# Autodesk Inventor assembly: 分析
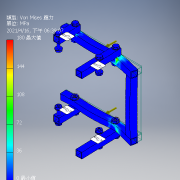
[picture p0: Inventor's stored thumbnail of the model, 180x180]
Saved by Autodesk Inventor 2019 (Build 230136000, 136)
## iProperties
Created: 2019-05-06
Part Number: 分析
Document SubType Name: Assembly
Designer: D03
Author: D03
## Documents named in this file (14)
- C:\Users\user\Desktop\分析.iam
- C:\Users\user\Desktop\新增資料夾\4.ipt
- C:\Users\user\Desktop\新增資料夾\3.ipt
- C:\Users\user\Desktop\新增資料夾\9.ipt
- C:\Users\user\Desktop\新增資料夾\CNS 150 - A - 2.2.ipt
- C:\Users\user\Desktop\新增資料夾\CNS 3128 - M 2 x 0.4.ipt
- C:\Users\user\Desktop\新增資料夾\CNS 3121 - M2 x 12.ipt
- C:\Users\user\Desktop\新增資料夾\2-1.ipt
- C:\Users\user\Desktop\分析\AIP\FEA\dksv0cvts.fins
- C:\Users\user\Desktop\分析\AIP\FEA\dksv0cvts.fsat
- C:\Users\user\Desktop\分析\AIP\FEA\dksv0cvuo.ftes
- C:\Users\user\Desktop\分析\AIP\FEA\dksv0cvuo.fwiz
- C:\Users\user\Desktop\分析\AIP\FEA\dksv0cvz4.fmsh
- C:\Users\user\Desktop\分析\AIP\FEA\dksv0cw00.fres
## Components (39 placed, 7 different names)
1. 3:1 — 插入:6, 插入:10, 插入:13, 插入:24, 貼合:47, 對稱:1, 齊平:22, 齊平:23
2. 3:2 — 插入:7, 插入:8, 插入:20, 插入:23, 貼合:48, 齊平:15, 齊平:16, 對稱:1
3. 4:1 — 插入:7, 插入:18, 插入:19
4. 4:2 — 插入:6, 插入:12, 插入:15
5. 9:1 — 插入:8, 插入:16, 插入:17
6. 9:2 — 插入:10, 插入:26, 插入:27
7. CNS 150 - A - 2.2:1 — 插入:15, 插入:50
8. CNS 150 - A - 2.2:2 — 插入:12, 插入:51
9. CNS 150 - A - 2.2:3 — 插入:24, 插入:36
10. CNS 150 - A - 2.2:4 — 插入:38
11. CNS 150 - A - 2.2:5 — 插入:20, 插入:40
12. CNS 150 - A - 2.2:6 — 插入:41
13. CNS 150 - A - 2.2:7 — 插入:19, 插入:52
14. CNS 150 - A - 2.2:8 — 插入:18, 插入:53
15. CNS 150 - A - 2.2:9 — 插入:26, 插入:48
16. CNS 150 - A - 2.2:10 — 插入:39
17. CNS 150 - A - 2.2:11 — 插入:27, 插入:49
18. CNS 150 - A - 2.2:12 — 插入:13, 插入:37
19. CNS 150 - A - 2.2:13 — 插入:23, 插入:43
20. CNS 150 - A - 2.2:14 — 插入:42
21. CNS 150 - A - 2.2:15 — 插入:17, 插入:54
22. CNS 150 - A - 2.2:16 — 插入:16, 插入:55
23. CNS 3128 - M 2 x 0.4:2 — 插入:39
24. CNS 3128 - M 2 x 0.4:3 — 插入:38
25. CNS 3128 - M 2 x 0.4:4 — 插入:37
26. CNS 3128 - M 2 x 0.4:5 — 插入:36
27. CNS 3128 - M 2 x 0.4:6 — 插入:42
28. CNS 3128 - M 2 x 0.4:7 — 插入:41
29. CNS 3128 - M 2 x 0.4:8 — 插入:43
30. CNS 3128 - M 2 x 0.4:9 — 插入:40
31. CNS 3121 - M2 x 12:1 — 插入:55
32. CNS 3121 - M2 x 12:2 — 插入:54
33. CNS 3121 - M2 x 12:3 — 插入:53
34. CNS 3121 - M2 x 12:4 — 插入:52
35. CNS 3121 - M2 x 12:5 — 插入:50
36. CNS 3121 - M2 x 12:6 — 插入:51
37. CNS 3121 - M2 x 12:7 — 插入:49
38. CNS 3121 - M2 x 12:8 — 插入:48
39. 2-1:2 — 貼合:47, 貼合:48, 齊平:15, 齊平:16, 齊平:22, 齊平:23, 齊平:26
## Relationships (47: Insert 32, Mate 9, Flush 5, Symmetry 1)
- 插入:6 [Insert]: 3:1 ↔ 4:2
- 插入:7 [Insert]: 3:2 ↔ 4:1
- 貼合:24 [Mate]
- 插入:8 [Insert]: 3:2 ↔ 9:1
- 插入:10 [Insert]: 3:1 ↔ 9:2
- 插入:12 [Insert]: 4:2 ↔ CNS 150 - A - 2.2:2
- 插入:13 [Insert]: 3:1 ↔ CNS 150 - A - 2.2:12
- 插入:15 [Insert]: 4:2 ↔ CNS 150 - A - 2.2:1
- 插入:16 [Insert]: 9:1 ↔ CNS 150 - A - 2.2:16
- 插入:17 [Insert]: 9:1 ↔ CNS 150 - A - 2.2:15
- 插入:18 [Insert]: 4:1 ↔ CNS 150 - A - 2.2:8
- 插入:19 [Insert]: 4:1 ↔ CNS 150 - A - 2.2:7
- 插入:20 [Insert]: 3:2 ↔ CNS 150 - A - 2.2:5
- 插入:23 [Insert]: 3:2 ↔ CNS 150 - A - 2.2:13
- 插入:24 [Insert]: 3:1 ↔ CNS 150 - A - 2.2:3
- 插入:26 [Insert]: 9:2 ↔ CNS 150 - A - 2.2:9
- 插入:27 [Insert]: 9:2 ↔ CNS 150 - A - 2.2:11
- 插入:36 [Insert]: CNS 150 - A - 2.2:3 ↔ CNS 3128 - M 2 x 0.4:5
- 插入:37 [Insert]: CNS 150 - A - 2.2:12 ↔ CNS 3128 - M 2 x 0.4:4
- 插入:38 [Insert]: CNS 150 - A - 2.2:4 ↔ CNS 3128 - M 2 x 0.4:3
- 插入:39 [Insert]: CNS 150 - A - 2.2:10 ↔ CNS 3128 - M 2 x 0.4:2
- 插入:40 [Insert]: CNS 150 - A - 2.2:5 ↔ CNS 3128 - M 2 x 0.4:9
- 插入:41 [Insert]: CNS 150 - A - 2.2:6 ↔ CNS 3128 - M 2 x 0.4:7
- 插入:42 [Insert]: CNS 150 - A - 2.2:14 ↔ CNS 3128 - M 2 x 0.4:6
- 插入:43 [Insert]: CNS 150 - A - 2.2:13 ↔ CNS 3128 - M 2 x 0.4:8
- 貼合:32 [Mate]
- 貼合:33 [Mate]
- 貼合:34 [Mate]
- 插入:48 [Insert]: CNS 150 - A - 2.2:9 ↔ CNS 3121 - M2 x 12:8
- 插入:49 [Insert]: CNS 150 - A - 2.2:11 ↔ CNS 3121 - M2 x 12:7
- 插入:50 [Insert]: CNS 150 - A - 2.2:1 ↔ CNS 3121 - M2 x 12:5
- 插入:51 [Insert]: CNS 150 - A - 2.2:2 ↔ CNS 3121 - M2 x 12:6
- 插入:52 [Insert]: CNS 150 - A - 2.2:7 ↔ CNS 3121 - M2 x 12:4
- 插入:53 [Insert]: CNS 150 - A - 2.2:8 ↔ CNS 3121 - M2 x 12:3
- 插入:54 [Insert]: CNS 150 - A - 2.2:15 ↔ CNS 3121 - M2 x 12:2
- 插入:55 [Insert]: CNS 150 - A - 2.2:16 ↔ CNS 3121 - M2 x 12:1
- 貼合:42 [Mate]
- 貼合:47 [Mate]: 3:1 ↔ 2-1:2
- 貼合:48 [Mate]: 3:2 ↔ 2-1:2
- 齊平:15 [Flush]: 3:2 ↔ 2-1:2
- 齊平:16 [Flush]: 3:2 ↔ 2-1:2
- 對稱:1 [Symmetry]: 3:1 ↔ 3:2
- 貼合:52 [Mate]
- 齊平:22 [Flush]: 3:1 ↔ 2-1:2
- 齊平:23 [Flush]: 3:1 ↔ 2-1:2
- 貼合:55 [Mate]
- 齊平:26 [Flush] (-2.5 mm): 2-1:2
## Named parameters: sa_0 = 1.1006e-09, sa_1 = -50000, sa_2 = -7.69e-11, sa_3 = 1.0947e-09, sa_4 = -50000, sa_5 = -7.69e-11
note: some values were not read from the file. Shown as the stored number, unit unknown: "sa_0", "sa_1", "sa_2", "sa_3", "sa_4", "sa_5".
